# Autodesk Inventor assembly: 前腕_1
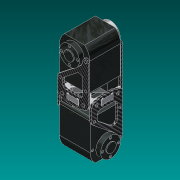
[picture p0: Inventor's stored thumbnail of the model, 180x180]
Saved by Autodesk Inventor 2016 (Build 200138000, 138)
## iProperties
Created: 2016-05-04
Part Number: 前腕_1
Document SubType Name: Assembly
Designer: hiroaki
Mass: 183.733 g
Surface Area: 334.039 cm^2
Volume: 106 cm^3
Density: 1.73333 g/cm^3
Author: hiroaki
## Documents named in this file (5)
- C:\Users\hiro\Documents\kenkyuu\二足\二足ver6.0\上半身\腕\上腕_1.iam
- C:\Users\hiro\Documents\kenkyuu\二足\二足ver6.0\既製品\B3M10xx.ipt
- C:\Users\hiro\Documents\kenkyuu\二足\二足ver6.0\既製品\free_horn.ipt
- C:\Users\hiro\Documents\kenkyuu\二足\二足ver6.0\上半身\腕\上腕_メインフレーム_1_1.ipt
- C:\Users\hiro\Documents\kenkyuu\二足\二足ver6.0\上半身\腕\上腕_サブフレーム_1_1.ipt
## Components (9 placed, 4 different names)
1. B3M11xx:1 — 挿入:1, 挿入:15, 挿入:16, 挿入:17, 挿入:20, 挿入:21
2. B3M11xx:2 — 挿入:2, 挿入:5, 挿入:6, 挿入:7, 挿入:10, 挿入:11, 挿入:12
3. free_horn:1 — 挿入:1
4. free_horn:2 — 挿入:2
5. 上腕_メインフレーム_1_1:1 — 挿入:3, 挿入:4, 挿入:8, 挿入:9, 挿入:13, 挿入:14, フラッシュ:1, フラッシュ:2, フラッシュ:3, 挿入:18, 挿入:19
6. 上腕_サブフレーム_1_1:1 — 挿入:8, 挿入:9, 挿入:10, 挿入:11, 挿入:12
7. 上腕_サブフレーム_1_1:2 — 挿入:3, 挿入:4, 挿入:5, 挿入:6, 挿入:7
8. 上腕_サブフレーム_1_1:3 — 挿入:18, 挿入:19, 挿入:20, 挿入:21
9. 上腕_サブフレーム_1_1:4 — 挿入:13, 挿入:14, 挿入:15, 挿入:16, 挿入:17
## Relationships (24: Insert 21, Flush 3)
- 挿入:1 [Insert]: B3M11xx:1 ↔ free_horn:1
- 挿入:2 [Insert]: B3M11xx:2 ↔ free_horn:2
- 挿入:3 [Insert]: 上腕_メインフレーム_1_1:1 ↔ 上腕_サブフレーム_1_1:2
- 挿入:4 [Insert]: 上腕_メインフレーム_1_1:1 ↔ 上腕_サブフレーム_1_1:2
- 挿入:5 [Insert]: B3M11xx:2 ↔ 上腕_サブフレーム_1_1:2
- 挿入:6 [Insert]: B3M11xx:2 ↔ 上腕_サブフレーム_1_1:2
- 挿入:7 [Insert]: B3M11xx:2 ↔ 上腕_サブフレーム_1_1:2
- 挿入:8 [Insert]: 上腕_メインフレーム_1_1:1 ↔ 上腕_サブフレーム_1_1:1
- 挿入:9 [Insert]: 上腕_メインフレーム_1_1:1 ↔ 上腕_サブフレーム_1_1:1
- 挿入:10 [Insert]: B3M11xx:2 ↔ 上腕_サブフレーム_1_1:1
- 挿入:11 [Insert]: B3M11xx:2 ↔ 上腕_サブフレーム_1_1:1
- 挿入:12 [Insert]: B3M11xx:2 ↔ 上腕_サブフレーム_1_1:1
- 挿入:13 [Insert]: 上腕_メインフレーム_1_1:1 ↔ 上腕_サブフレーム_1_1:4
- 挿入:14 [Insert]: 上腕_メインフレーム_1_1:1 ↔ 上腕_サブフレーム_1_1:4
- フラッシュ:1 [Flush]: 上腕_メインフレーム_1_1:1
- フラッシュ:2 [Flush]: 上腕_メインフレーム_1_1:1
- フラッシュ:3 [Flush]: 上腕_メインフレーム_1_1:1
- 挿入:15 [Insert]: B3M11xx:1 ↔ 上腕_サブフレーム_1_1:4
- 挿入:16 [Insert]: B3M11xx:1 ↔ 上腕_サブフレーム_1_1:4
- 挿入:17 [Insert]: B3M11xx:1 ↔ 上腕_サブフレーム_1_1:4
- 挿入:18 [Insert]: 上腕_メインフレーム_1_1:1 ↔ 上腕_サブフレーム_1_1:3
- 挿入:19 [Insert]: 上腕_メインフレーム_1_1:1 ↔ 上腕_サブフレーム_1_1:3
- 挿入:20 [Insert]: B3M11xx:1 ↔ 上腕_サブフレーム_1_1:3
- 挿入:21 [Insert]: B3M11xx:1 ↔ 上腕_サブフレーム_1_1:3
